# Autodesk Inventor assembly: Toughbox-mini-hex-long-turbocharge modification
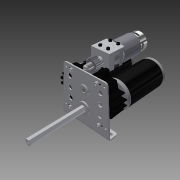
[picture p0: Inventor's stored thumbnail of the model, 180x180]
Saved by Autodesk Inventor 2013 (Build 170138000, 138)
## iProperties
Created: 2013-01-13
Part Number: Toughbox-mini-hex-long-turbocharge modification
Document SubType Name: Assembly
Designer: Moses
Mass: 4115.36 g
Surface Area: 2681.75 cm^2
Volume: 1070.7 cm^3
Density: 3.8436 g/cm^3
Translation Standard: STEP AP203
FileName: S:/Products/Gearboxes Spur Single Stage/Toughbox/Toughbox Mini/Toughbox-Mini.stp
PreProcessor: Unknown
PostProcessor: Build: 138, Release: 2013 RTM - Date: Thu 03/01/2012
Sent Units: millimeter
Uncertainty: 0.001
Author: Moses
## Documents named in this file (27)
- C:\Users\Moses\Documents\GitHub\frc2013CAD\Drivetrain\Toughbox-mini\Toughbox-mini-hex-long-turbocharge modification.iam
- C:\Users\Moses\Documents\GitHub\frc2013CAD\Drivetrain\Toughbox-mini\r6zz.ipt
- C:\Users\Moses\Documents\GitHub\frc2013CAD\Drivetrain\Toughbox-mini\Toughbox_d07.ipt
- C:\Users\Moses\Documents\GitHub\frc2013CAD\Drivetrain\Toughbox-mini\Toughbox_d05.ipt
- C:\Users\Moses\Documents\GitHub\frc2013CAD\Drivetrain\Toughbox-mini\Toughbox_d08.ipt
- C:\Users\Moses\Documents\GitHub\frc2013CAD\Drivetrain\Toughbox-mini\Toughbox_d06.ipt
- C:\Users\Moses\Documents\GitHub\frc2013CAD\Drivetrain\Toughbox-mini\fr-6-zz.ipt
- C:\Users\Moses\Documents\GitHub\frc2013CAD\Drivetrain\Toughbox-mini\10-32_nylock_nut.ipt
- C:\Users\Moses\Documents\GitHub\frc2013CAD\Drivetrain\Toughbox-mini\5-16_washer.ipt
- C:\Users\Moses\Documents\GitHub\frc2013CAD\Drivetrain\Toughbox-mini\Toughbox_d09.ipt
- C:\Users\Moses\Documents\GitHub\frc2013CAD\Drivetrain\Toughbox-mini\8mm_spring_clip.ipt
- C:\Users\Moses\Documents\GitHub\frc2013CAD\Drivetrain\Toughbox-mini\10-32x0625_shcs.ipt
- C:\Users\Moses\Documents\GitHub\frc2013CAD\Drivetrain\Toughbox-mini\CIM motor1.ipt
- C:\Users\Moses\Documents\GitHub\frc2013CAD\Drivetrain\Toughbox-mini\Toughbox_d31.ipt
- C:\Users\Moses\Documents\GitHub\frc2013CAD\Drivetrain\Toughbox-mini\fr8zz-hex.ipt
- C:\Users\Moses\Documents\GitHub\frc2013CAD\Drivetrain\Toughbox-mini\Toughbox-mini_d01-5-12 - turbocharge modification.ipt
- C:\Users\Moses\Documents\GitHub\frc2013CAD\Drivetrain\Toughbox-mini\Banebots P60\Banebots RS-775 P60 Planetary Gearbox 4  to 1 (0.5x1.5 shaft).iam
- C:\Users\Moses\Documents\GitHub\frc2013CAD\Drivetrain\Toughbox-mini\Banebots P60\AM-0129 Small Final Gear 20T.ipt
- C:\Users\Moses\Documents\GitHub\frc2013CAD\Drivetrain\Toughbox-mini\Banebots P60\Angle Aluminum P60 Mount.ipt
- C:\Users\Moses\Documents\GitHub\frc2013CAD\Drivetrain\Toughbox-mini\Banebots P60\Aluminum Spacer Part 1.ipt
- C:\Users\Moses\Documents\GitHub\frc2013CAD\Drivetrain\Toughbox-mini\Banebots P60\0.125 key.ipt
- C:\Users\Moses\Documents\GitHub\frc2013CAD\Drivetrain\Toughbox-mini\Banebots P60\10-32 Bolt.ipt
- C:\Users\Moses\Documents\GitHub\frc2013CAD\Drivetrain\Toughbox-mini\Banebots P60\Gearbox Hex Machine Screw 2.ipt
- C:\Users\Moses\Documents\GitHub\frc2013CAD\Drivetrain\Toughbox-mini\Banebots P60\Gearbox Hex Machine Screw.ipt
- C:\Users\Moses\Documents\GitHub\frc2013CAD\Drivetrain\Toughbox-mini\Banebots P60\Gearbox Hex Machine Screw 3.ipt
- C:\Users\Moses\Documents\GitHub\frc2013CAD\Drivetrain\Toughbox-mini\Banebots P60\Aluminum Spacer Part 2.ipt
- C:\Users\Moses\Documents\GitHub\frc2013CAD\Drivetrain\Toughbox-mini\Toughbox-mini_d02.ipt
## Components (52 placed, 26 different names)
1. r6zz:1
2. r6zz:2 — Mate:2, Mate:1
3. Toughbox_d31:1 — Mate:1, Mate:2
4. Toughbox_d07:1
5. Toughbox_d05:1
6. Toughbox_d08:1
7. Toughbox_d06:1
8. fr-6-zz:1 — Mate:4
9. fr8zz-hex:1
10. 10-32_nylock_nut:1
11. 10-32_nylock_nut:2
12. 10-32_nylock_nut:3 — Insert:9
13. 10-32_nylock_nut:4 — Insert:8
14. 5-16_washer:1
15. 5-16_washer:2
16. 5-16_washer:3
17. 5-16_washer:4
18. Toughbox_d09:1
19. Toughbox_d09:2
20. 8mm_spring_clip:1
21. 8mm_spring_clip:2
22. Toughbox-mini_d01-5-12 - turbocharge modification:1 — Insert:1, Insert:2, Insert:8, Insert:9, Mate:5, Mate:6, Mate:7, Insert:13, Insert:14, Insert:20, Insert:21, Mate:15, Mate:16, Mate:17
23. 10-32x0625_shcs:1
24. 10-32x0625_shcs:2
25. 10-32x0625_shcs:3
26. 10-32x0625_shcs:4
27. 10-32x0625_shcs:5
28. 10-32x0625_shcs:6
29. 10-32x0625_shcs:7
30. 10-32x0625_shcs:8
31. CIM motor1:1 — Insert:1
32. CIM motor1:2 — Insert:2
33. Banebots RS-775 P60 Planetary Gearbox 4  to 1 (0.5x1.5 shaft):1 [sub-assembly] — Mate:4, Mate:8, Flush:1, Mate:9, Mate:10, Flush:2, Mate:11, Flush:3, Mate:13, Mate:14, Insert:10, Insert:11, Insert:12, Insert:19, Mate:18, Mate:19
34. AM-0129 Small Final Gear 20T:1 — Flush:1, Mate:11, Mate:12, Flush:3
35. Angle Aluminum P60 Mount:1 — Mate:5, Mate:6, Mate:7, Mate:8, Insert:15, Insert:16, Insert:17, Insert:18, Insert:22, Insert:23, Mate:19
36. 0.125 key:1 — Mate:9, Mate:10, Flush:2, Mate:12
37. Aluminum Spacer Part 1:1 — Mate:13, Mate:14
38. 10-32 Bolt:1 — Insert:10
39. Gearbox Hex Machine Screw 2:1 — Insert:11, Mate:18
40. Gearbox Hex Machine Screw 2:2 — Insert:12
41. Gearbox Hex Machine Screw:1 — Insert:13
42. Gearbox Hex Machine Screw:2 — Insert:14
43. Gearbox Hex Machine Screw 3:1 — Insert:15
44. Gearbox Hex Machine Screw 3:2 — Insert:16
45. Gearbox Hex Machine Screw 3:3 — Insert:18
46. Gearbox Hex Machine Screw 3:4 — Insert:17
47. Aluminum Spacer Part 2:1 — Insert:19
48. 10-32x0625_shcs:9 — Insert:20
49. 10-32x0625_shcs:10 — Insert:21
50. 10-32_nylock_nut:5 — Insert:23
51. 10-32_nylock_nut:6 — Insert:22
52. Toughbox-mini_d02:1 — Mate:15, Mate:16, Mate:17
## Relationships (39: Insert 18, Mate 18, Flush 3)
- Insert:1: Toughbox-mini_d01-5-12 - turbocharge modification:1 ↔ CIM motor1:1
- Insert:2: Toughbox-mini_d01-5-12 - turbocharge modification:1 ↔ CIM motor1:2
- Mate:1: r6zz:2 ↔ Toughbox_d31:1
- Mate:2: r6zz:2 ↔ Toughbox_d31:1
- Insert:8: 10-32_nylock_nut:4 ↔ Toughbox-mini_d01-5-12 - turbocharge modification:1
- Insert:9: 10-32_nylock_nut:3 ↔ Toughbox-mini_d01-5-12 - turbocharge modification:1
- Mate:4 (44.45 mm): fr-6-zz:1 ↔ Banebots RS-775 P60 Planetary Gearbox 4  to 1 (0.5x1.5 shaft):1
- Mate:5: Toughbox-mini_d01-5-12 - turbocharge modification:1 ↔ Angle Aluminum P60 Mount:1
- Mate:6: Toughbox-mini_d01-5-12 - turbocharge modification:1 ↔ Angle Aluminum P60 Mount:1
- Mate:7: Toughbox-mini_d01-5-12 - turbocharge modification:1 ↔ Angle Aluminum P60 Mount:1
- Mate:8: Banebots RS-775 P60 Planetary Gearbox 4  to 1 (0.5x1.5 shaft):1 ↔ Angle Aluminum P60 Mount:1
- Flush:1: Banebots RS-775 P60 Planetary Gearbox 4  to 1 (0.5x1.5 shaft):1 ↔ AM-0129 Small Final Gear 20T:1
- Mate:9: Banebots RS-775 P60 Planetary Gearbox 4  to 1 (0.5x1.5 shaft):1 ↔ 0.125 key:1
- Mate:10: Banebots RS-775 P60 Planetary Gearbox 4  to 1 (0.5x1.5 shaft):1 ↔ 0.125 key:1
- Flush:2: Banebots RS-775 P60 Planetary Gearbox 4  to 1 (0.5x1.5 shaft):1 ↔ 0.125 key:1
- Mate:11: Banebots RS-775 P60 Planetary Gearbox 4  to 1 (0.5x1.5 shaft):1 ↔ AM-0129 Small Final Gear 20T:1
- Mate:12: AM-0129 Small Final Gear 20T:1 ↔ 0.125 key:1
- Flush:3 (12.7 mm): Banebots RS-775 P60 Planetary Gearbox 4  to 1 (0.5x1.5 shaft):1 ↔ AM-0129 Small Final Gear 20T:1
- Mate:13: Banebots RS-775 P60 Planetary Gearbox 4  to 1 (0.5x1.5 shaft):1 ↔ Aluminum Spacer Part 1:1
- Mate:14: Banebots RS-775 P60 Planetary Gearbox 4  to 1 (0.5x1.5 shaft):1 ↔ Aluminum Spacer Part 1:1
- Insert:10: Banebots RS-775 P60 Planetary Gearbox 4  to 1 (0.5x1.5 shaft):1 ↔ 10-32 Bolt:1
- Insert:11: Banebots RS-775 P60 Planetary Gearbox 4  to 1 (0.5x1.5 shaft):1 ↔ Gearbox Hex Machine Screw 2:1
- Insert:12: Banebots RS-775 P60 Planetary Gearbox 4  to 1 (0.5x1.5 shaft):1 ↔ Gearbox Hex Machine Screw 2:2
- Insert:13: Toughbox-mini_d01-5-12 - turbocharge modification:1 ↔ Gearbox Hex Machine Screw:1
- Insert:14: Toughbox-mini_d01-5-12 - turbocharge modification:1 ↔ Gearbox Hex Machine Screw:2
- Insert:15: Angle Aluminum P60 Mount:1 ↔ Gearbox Hex Machine Screw 3:1
- Insert:16: Angle Aluminum P60 Mount:1 ↔ Gearbox Hex Machine Screw 3:2
- Insert:17: Angle Aluminum P60 Mount:1 ↔ Gearbox Hex Machine Screw 3:4
- Insert:18: Angle Aluminum P60 Mount:1 ↔ Gearbox Hex Machine Screw 3:3
- Insert:19: Banebots RS-775 P60 Planetary Gearbox 4  to 1 (0.5x1.5 shaft):1 ↔ Aluminum Spacer Part 2:1
- Insert:20: Toughbox-mini_d01-5-12 - turbocharge modification:1 ↔ 10-32x0625_shcs:9
- Insert:21: Toughbox-mini_d01-5-12 - turbocharge modification:1 ↔ 10-32x0625_shcs:10
- Insert:22: Angle Aluminum P60 Mount:1 ↔ 10-32_nylock_nut:6
- Insert:23: Angle Aluminum P60 Mount:1 ↔ 10-32_nylock_nut:5
- Mate:15: Toughbox-mini_d01-5-12 - turbocharge modification:1 ↔ Toughbox-mini_d02:1
- Mate:16: Toughbox-mini_d01-5-12 - turbocharge modification:1 ↔ Toughbox-mini_d02:1
- Mate:17: Toughbox-mini_d01-5-12 - turbocharge modification:1 ↔ Toughbox-mini_d02:1
- Mate:18: Banebots RS-775 P60 Planetary Gearbox 4  to 1 (0.5x1.5 shaft):1 ↔ Gearbox Hex Machine Screw 2:1
- Mate:19: Banebots RS-775 P60 Planetary Gearbox 4  to 1 (0.5x1.5 shaft):1 ↔ Angle Aluminum P60 Mount:1
